# Autodesk Inventor assembly: YaxisNew
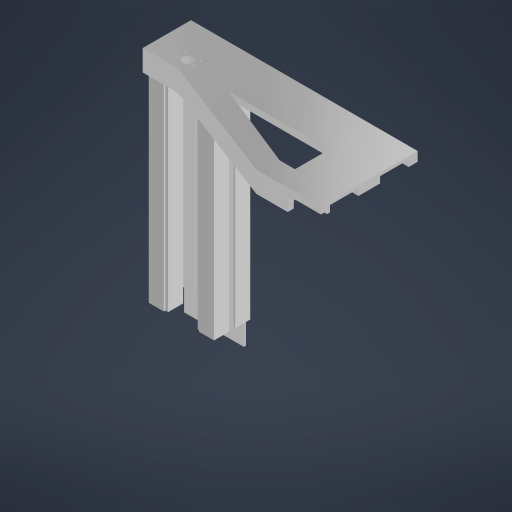
[picture p0: Inventor's stored thumbnail of the model, 512x512]
Saved by Autodesk Inventor 2024 (Build 280153000, 153)
## iProperties
Created: 2023-06-18
Part Number: YaxisNew
Document SubType Name: Assembly
Designer: KirikDK
Mass: 23414.9 g
Surface Area: 24958.2 cm^2
Volume: 9928.3 cm^3
Density: 2.3584 g/cm^3
Author: KirikDK
## Documents named in this file (5)
- C:\Users\KirikDK\Documents\Stanok2023\YaxisNew.iam
- C:\Users\KirikDK\Documents\Stanok2023\YflanecSborka.iam
- C:\Users\KirikDK\Documents\Stanok2023\YaxisUgolok.ipt
- C:\Users\KirikDK\Documents\Stanok2023\BackYflanec.ipt
- C:\Users\KirikDK\Documents\Stanok2023\YKrep.ipt
## Components (10 placed, 4 different names)
1. YflanecSborka:1 [sub-assembly] — Mate:1, Flush:1, Flush:2, Mate:2, Mate:3, Flush:3, Mate:4, Flush:4, Flush:5, Mate:5, Mate:6, Flush:6, Mate:10, Mate:12, Mate:15, Mate:16, Mate:21
2. YaxisUgolok:1 — Mate:2, Mate:3, Flush:3, Mate:7, Mate:8, Mate:11
3. YaxisUgolok:2 — Mate:5, Mate:6, Flush:6
4. YaxisUgolok:4 — Mate:4, Flush:4, Flush:5, Mate:17, Mate:18
5. YaxisUgolok:5 — Mate:1, Flush:1, Flush:2, Mate:14
6. BackYflanec:2 — Mate:9, Mate:10, Mate:11
7. YKrep:1 — Mate:7, Mate:8, Mate:9, Mate:12, Mate:13
8. YaxisUgolok:6 — Mate:13, Mate:14, Mate:15
9. YKrep:3 — Mate:16, Mate:17, Mate:18, Mate:19, Mate:20
10. YaxisUgolok:7 — Mate:19, Mate:20, Mate:21
## Relationships (27: Mate 21, Flush 6)
- Mate:1: YflanecSborka:1 ↔ YaxisUgolok:5
- Flush:1: YflanecSborka:1 ↔ YaxisUgolok:5
- Flush:2: YflanecSborka:1 ↔ YaxisUgolok:5
- Mate:2: YflanecSborka:1 ↔ YaxisUgolok:1
- Mate:3: YflanecSborka:1 ↔ YaxisUgolok:1
- Flush:3: YflanecSborka:1 ↔ YaxisUgolok:1
- Mate:4: YflanecSborka:1 ↔ YaxisUgolok:4
- Flush:4: YflanecSborka:1 ↔ YaxisUgolok:4
- Flush:5: YflanecSborka:1 ↔ YaxisUgolok:4
- Mate:5: YflanecSborka:1 ↔ YaxisUgolok:2
- Mate:6: YflanecSborka:1 ↔ YaxisUgolok:2
- Flush:6: YflanecSborka:1 ↔ YaxisUgolok:2
- Mate:7: YaxisUgolok:1 ↔ YKrep:1
- Mate:8: YaxisUgolok:1 ↔ YKrep:1
- Mate:9: BackYflanec:2 ↔ YKrep:1
- Mate:10: YflanecSborka:1 ↔ BackYflanec:2
- Mate:11: YaxisUgolok:1 ↔ BackYflanec:2
- Mate:12: YflanecSborka:1 ↔ YKrep:1
- Mate:13: YKrep:1 ↔ YaxisUgolok:6
- Mate:14: YaxisUgolok:5 ↔ YaxisUgolok:6
- Mate:15: YflanecSborka:1 ↔ YaxisUgolok:6
- Mate:16: YflanecSborka:1 ↔ YKrep:3
- Mate:17: YaxisUgolok:4 ↔ YKrep:3
- Mate:18: YaxisUgolok:4 ↔ YKrep:3
- Mate:19: YKrep:3 ↔ YaxisUgolok:7
- Mate:20: YKrep:3 ↔ YaxisUgolok:7
- Mate:21: YflanecSborka:1 ↔ YaxisUgolok:7
